# Autodesk Inventor assembly: ASY ANP 1425 FDS way 5
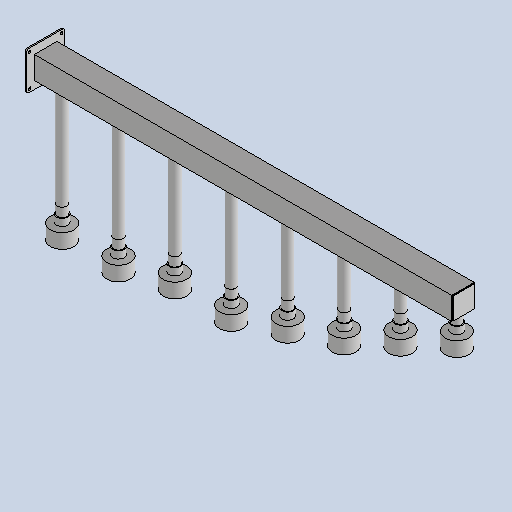
[picture p0: Inventor's stored thumbnail of the model, 512x512]
Saved by Autodesk Inventor 2025 (Build 290162010, 162A)
## iProperties
Created: 2025-07-02
Part Number: ASY ANP 1425 FDS way 5
Document SubType Name: Assembly
Designer: admin
Author: user
## Documents named in this file (11)
- C:\Users\pokla\Documents\Inventor\ANP--Antipayuta\FDS 1400\ASY ANP 1425 FDS way 5.iam
- C:\Users\pokla\Documents\Inventor\ANP--Antipayuta\FDS 1400\ANP 1435 FDS WAY tube5.ipt
- C:\Users\pokla\Documents\Inventor\ANP--Antipayuta\FDS 1400\ANP 1425 FDS Way FLANGE.ipt
- C:\Users\pokla\Documents\Inventor\ANP--Antipayuta\FDS 1400\ANP 1426 FDS way cup.ipt
- C:\Users\pokla\Documents\Inventor\ANP--Antipayuta\FDS 1400\ANP dummy filter element.ipt
- C:\Users\pokla\Documents\Inventor\ANP--Antipayuta\FDS 1400\ANP dummy pipe nippel.ipt
- C:\Users\pokla\Documents\Inventor\ANP--Antipayuta\FDS 1400\ANP 1446 FDS thread  tube6.ipt
- C:\Users\pokla\Documents\Inventor\ANP--Antipayuta\FDS 1400\ANP 1447 FDS thread  tube7.ipt
- C:\Users\pokla\Documents\Inventor\ANP--Antipayuta\FDS 1400\ANP 1448 FDS thread  tube8.ipt
- C:\Users\pokla\Documents\Inventor\ANP--Antipayuta\FDS 1400\ANP 1449 FDS thread  tube9.ipt
- C:\Users\pokla\Documents\Inventor\ANP--Antipayuta\FDS 1400\ANP 1451 FDS thread  tube10.ipt
## Components (26 placed, 10 different names)
1. TKS 3535 FDS WAY tube5:1 — Rigid:34, Rigid:35, Rigid:36, Rigid:51, Rigid:52, Rigid:53, Rigid:54, Rigid:55, Rigid:39, Rigid:31
2. TKS 3525 FDS Way FLANGE:1 — Rigid:34
3. TKS 3526 FDS way cup:1 — Rigid:35
4. TKS dummy filter element:1 — Rigid:1
5. TKS dummy pipe nippel:1 — Rigid:1, Rigid:44
6. TKS dummy filter element:2 — Rigid:6
7. TKS dummy pipe nippel:2 — Rigid:6, Rigid:46
8. TKS dummy filter element:3 — Rigid:11
9. TKS dummy pipe nippel:3 — Rigid:11, Rigid:47
10. TKS dummy filter element:4 — Rigid:14
11. TKS dummy pipe nippel:4 — Rigid:14, Rigid:45
12. TKS dummy filter element:5 — Rigid:27
13. TKS dummy pipe nippel:5 — Rigid:27, Rigid:48
14. TKS dummy filter element:6 — Rigid:33
15. TKS dummy pipe nippel:6 — Rigid:33, Rigid:36
16. TKS 3546 FDS thread  tube6:1 — Rigid:48, Rigid:51
17. TKS 3547 FDS thread  tube7:1 — Rigid:47, Rigid:52
18. TKS 3548 FDS thread  tube8:1 — Rigid:46, Rigid:53
19. TKS 3549 FDS thread  tube9:1 — Rigid:45, Rigid:54
20. TKS 3551 FDS thread  tube10:1 — Rigid:44, Rigid:55
21. TKS dummy filter element:7 — Rigid:37
22. TKS dummy pipe nippel:7 — Rigid:37, Rigid:38
23. TKS 3546 FDS thread  tube6:2 — Rigid:39, Rigid:38
24. TKS dummy filter element:8
25. TKS dummy pipe nippel:8
26. TKS 3547 FDS thread  tube7:2 — Rigid:31
## Relationships (25: WeldJoint 25)
- Rigid:34 [WeldJoint] (2 mm): TKS 3535 FDS WAY tube5:1 ↔ TKS 3525 FDS Way FLANGE:1
- Rigid:35 [WeldJoint]: TKS 3535 FDS WAY tube5:1 ↔ TKS 3526 FDS way cup:1
- Rigid:1 [WeldJoint]: TKS dummy filter element:1 ↔ TKS dummy pipe nippel:1
- Rigid:6 [WeldJoint]: TKS dummy filter element:2 ↔ TKS dummy pipe nippel:2
- Rigid:11 [WeldJoint]: TKS dummy filter element:3 ↔ TKS dummy pipe nippel:3
- Rigid:14 [WeldJoint]: TKS dummy filter element:4 ↔ TKS dummy pipe nippel:4
- Rigid:27 [WeldJoint]: TKS dummy filter element:5 ↔ TKS dummy pipe nippel:5
- Rigid:33 [WeldJoint]: TKS dummy filter element:6 ↔ TKS dummy pipe nippel:6
- Rigid:36 [WeldJoint]: TKS 3535 FDS WAY tube5:1 ↔ TKS dummy pipe nippel:6
- Rigid:48 [WeldJoint]: TKS dummy pipe nippel:5 ↔ TKS 3546 FDS thread  tube6:1
- Rigid:51 [WeldJoint]: TKS 3535 FDS WAY tube5:1 ↔ TKS 3546 FDS thread  tube6:1
- Rigid:47 [WeldJoint]: TKS dummy pipe nippel:3 ↔ TKS 3547 FDS thread  tube7:1
- Rigid:52 [WeldJoint]: TKS 3535 FDS WAY tube5:1 ↔ TKS 3547 FDS thread  tube7:1
- Rigid:46 [WeldJoint]: TKS dummy pipe nippel:2 ↔ TKS 3548 FDS thread  tube8:1
- Rigid:53 [WeldJoint]: TKS 3535 FDS WAY tube5:1 ↔ TKS 3548 FDS thread  tube8:1
- Rigid:45 [WeldJoint]: TKS dummy pipe nippel:4 ↔ TKS 3549 FDS thread  tube9:1
- Rigid:54 [WeldJoint]: TKS 3535 FDS WAY tube5:1 ↔ TKS 3549 FDS thread  tube9:1
- Rigid:44 [WeldJoint]: TKS dummy pipe nippel:1 ↔ TKS 3551 FDS thread  tube10:1
- Rigid:55 [WeldJoint]: TKS 3535 FDS WAY tube5:1 ↔ TKS 3551 FDS thread  tube10:1
- Rigid:37 [WeldJoint]: TKS dummy filter element:7 ↔ TKS dummy pipe nippel:7
- Rigid:39 [WeldJoint]: TKS 3535 FDS WAY tube5:1 ↔ TKS 3546 FDS thread  tube6:2
- Rigid:38 [WeldJoint]: TKS dummy pipe nippel:7 ↔ TKS 3546 FDS thread  tube6:2
- [WeldJoint]: TKS dummy filter element:8 ↔ TKS dummy pipe nippel:8
- [WeldJoint]: TKS dummy pipe nippel:8 ↔ TKS 3547 FDS thread  tube7:2
- Rigid:31 [WeldJoint]: TKS 3535 FDS WAY tube5:1 ↔ TKS 3547 FDS thread  tube7:2
## Named parameters: d28_d14 = 0 mm, d29_d4 = 0 mm
